# Autodesk Inventor assembly: NUCBase-PCB
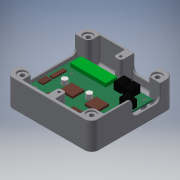
[picture p0: Inventor's stored thumbnail of the model, 180x180]
Saved by Autodesk Inventor 2016 (Build 200138000, 138)
## iProperties
Created: 2015-09-25
Part Number: NUCBase-PCB
Document SubType Name: Assembly
Designer: lachesis
Author: lachesis
## Documents named in this file (3)
- C:\Users\lachesis\git\Swarmie-Build\Swarmie-Assembly\Assemblies\NUCBase-PCB.iam
- C:\Users\lachesis\git\Swarmie-Build\Swarmie-Assembly\Parts\NUCBasePCB.ipt
- C:\Users\lachesis\git\Swarmie-Build\Swarmie-Assembly\Parts\PCB.ipt
## Components (2 placed, 2 different names)
1. NUCBasePCB:1 — Rigid:1
2. PCB:1 — Rigid:1
## Relationships (1: WeldJoint 1)
- Rigid:1 [WeldJoint]: NUCBasePCB:1 ↔ PCB:1
